# Autodesk Inventor assembly: Double sided license plate no cover
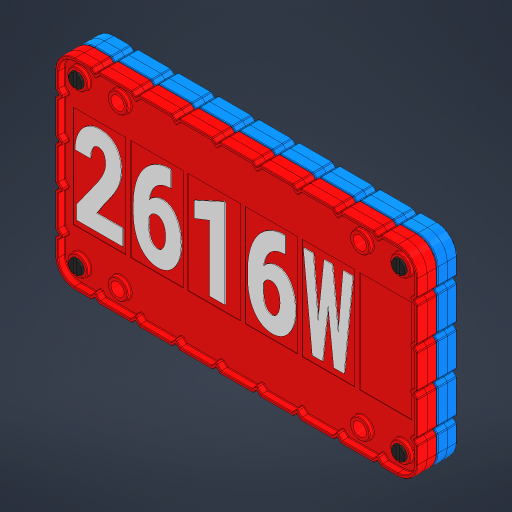
[picture p0: Inventor's stored thumbnail of the model, 512x512]
Saved by Autodesk Inventor 2023.2 (Build 272271030, 271C)
## iProperties
Created: 2022-06-18
Part Number: Double sided license plate no cover
Document SubType Name: Assembly
Designer: Main Account
Author: Main Account
## Documents named in this file (6)
- C:\Users\Main Account\InventorProjects\VEX\Custom Library\Double sided license plate no cover.iam
- C:\Users\Main Account\InventorProjects\VEX\Library Backup\Library 1.4\Structure\Hardware\VEX IQ Pin.ipt
- C:\Users\Main Account\InventorProjects\VEX\Custom Library\License Plate Numbers.ipt
- License Plate Numbers.ipt
- C:\Users\Main Account\InventorProjects\VEX\Library Backup\Library 1.4\Miscellaneous\Blue License Plate.ipt
- C:\Users\Main Account\InventorProjects\VEX\Library Backup\Library 1.4\Miscellaneous\Red License Plate.ipt
## Components (8 placed, 4 different names)
1. Red License Plate:2
2. Blue License Plate:1 — Insert:5, Insert:6, Insert:7, Insert:8, Mate:9, Mate:10, Mate:11
3. VEX IQ Pin:1 — Insert:5
4. VEX IQ Pin:2 — Insert:8
5. VEX IQ Pin:3 — Insert:7
6. VEX IQ Pin:4 — Insert:6
7. License Plate Numbers:1
8. License Plate Numbers:2 — Mate:9, Mate:10, Mate:11
## Relationships (14: Insert 8, Mate 6)
- [Insert]: Red License Plate:2 ↔ VEX IQ Pin:3
- [Insert]: Red License Plate:2 ↔ VEX IQ Pin:1
- [Insert]: Red License Plate:2 ↔ VEX IQ Pin:2
- [Insert]: Red License Plate:2 ↔ VEX IQ Pin:4
- Insert:5: Blue License Plate:1 ↔ VEX IQ Pin:1
- Insert:6: Blue License Plate:1 ↔ VEX IQ Pin:4
- Insert:7: Blue License Plate:1 ↔ VEX IQ Pin:3
- Insert:8: Blue License Plate:1 ↔ VEX IQ Pin:2
- [Mate]: Red License Plate:2 ↔ License Plate Numbers:1
- [Mate]: Red License Plate:2 ↔ License Plate Numbers:1
- [Mate]: Red License Plate:2 ↔ License Plate Numbers:1
- Mate:9: Blue License Plate:1 ↔ License Plate Numbers:2
- Mate:10: Blue License Plate:1 ↔ License Plate Numbers:2
- Mate:11: Blue License Plate:1 ↔ License Plate Numbers:2
